# Autodesk Inventor assembly: PowerPlugBlock
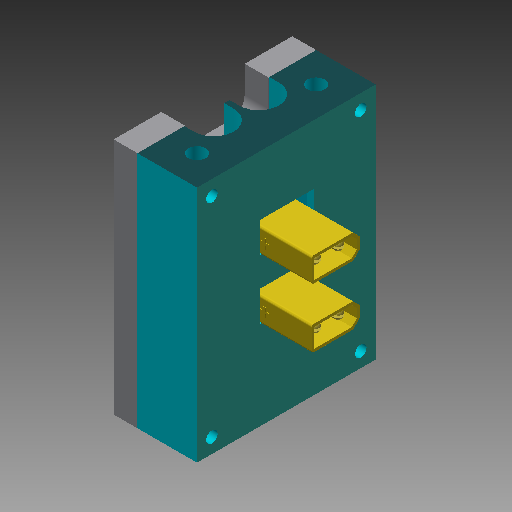
[picture p0: Inventor's stored thumbnail of the model, 512x512]
Saved by Autodesk Inventor 2019 (Build 230136000, 136)
## iProperties
Created: 2020-04-21
Part Number: PowerPlugBlock
Document SubType Name: Assembly
Designer: james
Author: james
## Documents named in this file (5)
- F:\JimsRobot\FIRSTRobots\Design\TornadoPlatypus\PowerPlugBlock.iam
- F:\JimsRobot\FIRSTRobots\Design\Library\RevRobotics\XT30_Stecker.ipt
- F:\JimsRobot\FIRSTRobots\Design\TornadoPlatypus\PowerPlugBlock.ipt
- F:\JimsRobot\FIRSTRobots\Design\TornadoPlatypus\PowerWire.ipt
- F:\JimsRobot\FIRSTRobots\Design\TornadoPlatypus\PowerPlugBlockBack.ipt
## Components (8 placed, 4 different names)
1. XT30_Stecker:1 — Mate:5, Mate:6, Mate:7, Mate:8, Mate:10, Mate:11, Mate:13
2. XT30_Stecker:2 — Mate:1, Mate:2, Mate:3, Mate:4, Mate:9, Mate:12, Mate:14
3. PowerPlugBlock:1 — Mate:9, Mate:10, Mate:11, Mate:12, Mate:13, Mate:14, Mate:15, Flush:1, Flush:2
4. PowerWire:1 — Mate:1, Mate:4
5. PowerWire:2 — Mate:2, Mate:3
6. PowerWire:3 — Mate:5, Mate:8
7. PowerWire:4 — Mate:6, Mate:7
8. PowerPlugBlockBack:1 — Mate:15, Flush:1, Flush:2
## Relationships (17: Mate 15, Flush 2)
- Mate:1: XT30_Stecker:2 ↔ PowerWire:1
- Mate:2: XT30_Stecker:2 ↔ PowerWire:2
- Mate:3: XT30_Stecker:2 ↔ PowerWire:2
- Mate:4: XT30_Stecker:2 ↔ PowerWire:1
- Mate:5: XT30_Stecker:1 ↔ PowerWire:3
- Mate:6: XT30_Stecker:1 ↔ PowerWire:4
- Mate:7: XT30_Stecker:1 ↔ PowerWire:4
- Mate:8: XT30_Stecker:1 ↔ PowerWire:3
- Mate:9: XT30_Stecker:2 ↔ PowerPlugBlock:1
- Mate:10: XT30_Stecker:1 ↔ PowerPlugBlock:1
- Mate:11: XT30_Stecker:1 ↔ PowerPlugBlock:1
- Mate:12: XT30_Stecker:2 ↔ PowerPlugBlock:1
- Mate:13: XT30_Stecker:1 ↔ PowerPlugBlock:1
- Mate:14: XT30_Stecker:2 ↔ PowerPlugBlock:1
- Mate:15: PowerPlugBlock:1 ↔ PowerPlugBlockBack:1
- Flush:1: PowerPlugBlock:1 ↔ PowerPlugBlockBack:1
- Flush:2: PowerPlugBlock:1 ↔ PowerPlugBlockBack:1
